# Autodesk Inventor assembly: XEndRight
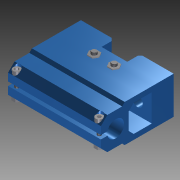
[picture p0: Inventor's stored thumbnail of the model, 180x180]
Saved by Autodesk Inventor 2015 (Build 190159000, 159)
## iProperties
Created: 2014-08-16
Part Number: XEndRight
Document SubType Name: Assembly
Designer: Jack
Author: Jack
## Documents named in this file (11)
- C:\Users\Jack\ownCloud\Projects\CoreXY\InventorModel\XAxis\DualE3DXEnd\XEndRight.iam
- C:\Users\Jack\ownCloud\Projects\CoreXY\InventorModel\XAxis\DualE3DXEnd\XEnd.ipt
- C:\Users\Jack\ownCloud\Projects\CoreXY\InventorModel\Hardware\Nuts\Nut3.ipt
- C:\Users\Jack\ownCloud\Projects\CoreXY\InventorModel\Hardware\Bolts\SHCS\SHCS3\SHCS3x18.ipt
- C:\Users\Jack\ownCloud\Projects\CoreXY\InventorModel\Hardware\Bolts\SHCS\SHCS4\SHCS4x30.ipt
- C:\Users\Jack\ownCloud\Projects\CoreXY\InventorModel\Hardware\Nuts\Nut4.ipt
- C:\Users\Jack\ownCloud\Projects\CoreXY\InventorModel\Hardware\Bearing\BearingRadialBall\BearingRadialBallF624zz.ipt
- C:\Users\Jack\ownCloud\Projects\CoreXY\InventorModel\Hardware\Wahsers\M4Washer.ipt
- C:\Users\Jack\ownCloud\Projects\CoreXY\InventorModel\Hardware\Bolts\SHCS\SHCS3\SHCS3x8.ipt
- C:\Users\Jack\ownCloud\Projects\CoreXY\InventorModel\XAxis\DualE3DXEnd\XAxisBearingSpacer.ipt
- C:\Users\Jack\ownCloud\Projects\CoreXY\InventorModel\Hardware\Bearing\BearingLinear\BearingLinearLMK8.ipt
## Components (25 placed, 10 different names)
1. XEnd:1 — Mate:5, Mate:6, Mate:7, Mate:8, Mate:9, Angle:1, Angle:2, Mate:10, Mate:11, Mate:13, Mate:15, Mate:16, Mate:17, Mate:18, Mate:19, Angle:3, Angle:4, Mate:22, Mate:23, Mate:40, Mate:41, Angle:5, Angle:6, Mate:44, Mate:45, Mate:46, Mate:47, Mate:62, Mate:63, Flush:3, Flush:4
2. XAxisBearingSpacer:1 — Mate:52, Mate:53
3. XAxisBearingSpacer:2 — Mate:54, Mate:55
4. BearingRadialBallF624zz:3
5. BearingRadialBallF624zz:4 — Mate:60, Mate:61
6. BearingLinearLMK8:1 — Mate:62, Flush:3
7. BearingLinearLMK8:2 — Mate:63, Flush:4
8. BearingRadialBallF624zz:1
9. BearingRadialBallF624zz:2
10. M4Washer:4 — Mate:38, Mate:46
11. M4Washer:3 — Mate:53, Mate:61
12. M4Washer:2 — Mate:30, Mate:55
13. M4Washer:1 — Mate:47
14. Nut4:2 — Mate:21, Angle:4, Mate:23
15. Nut4:1 — Mate:20, Angle:3, Mate:22
16. SHCS4x30:2 — Mate:17, Mate:18, Mate:20, Mate:38, Mate:52, Mate:60
17. SHCS4x30:1 — Mate:16, Mate:19, Mate:21, Mate:30, Mate:54
18. Nut3:3 — Mate:43, Angle:6, Mate:45, Flush:1
19. Nut3:4 — Mate:42, Angle:5, Mate:44, Flush:2
20. SHCS3x8:1 — Mate:40, Mate:42, Flush:2
21. SHCS3x8:2 — Mate:41, Mate:43, Flush:1
22. SHCS3x18:2 — Mate:14, Mate:15
23. SHCS3x18:1 — Mate:12, Mate:13
24. Nut3:2 — Mate:8, Angle:1, Mate:11, Mate:12
25. Nut3:1 — Mate:9, Angle:2, Mate:10, Mate:14
## Relationships (55: Mate 45, Angle 6, Flush 4)
- Mate:5: XEnd:1
- Mate:6: XEnd:1
- Mate:7: XEnd:1
- Mate:8: XEnd:1 ↔ Nut3:2
- Mate:9: XEnd:1 ↔ Nut3:1
- Angle:1 (0 deg): XEnd:1 ↔ Nut3:2
- Angle:2 (0 deg): XEnd:1 ↔ Nut3:1
- Mate:10: XEnd:1 ↔ Nut3:1
- Mate:11: XEnd:1 ↔ Nut3:2
- Mate:12: SHCS3x18:1 ↔ Nut3:2
- Mate:13: XEnd:1 ↔ SHCS3x18:1
- Mate:14: SHCS3x18:2 ↔ Nut3:1
- Mate:15: XEnd:1 ↔ SHCS3x18:2
- Mate:16: XEnd:1 ↔ SHCS4x30:1
- Mate:17: XEnd:1 ↔ SHCS4x30:2
- Mate:18: XEnd:1 ↔ SHCS4x30:2
- Mate:19: XEnd:1 ↔ SHCS4x30:1
- Mate:20: Nut4:1 ↔ SHCS4x30:2
- Mate:21: Nut4:2 ↔ SHCS4x30:1
- Angle:3 (0 deg): XEnd:1 ↔ Nut4:1
- Angle:4 (0 deg): XEnd:1 ↔ Nut4:2
- Mate:22: XEnd:1 ↔ Nut4:1
- Mate:23: XEnd:1 ↔ Nut4:2
- [Mate]: BearingRadialBallF624zz:1 ↔ BearingRadialBallF624zz:2
- [Mate]: BearingRadialBallF624zz:1 ↔ BearingRadialBallF624zz:2
- [Mate]: BearingRadialBallF624zz:1 ↔ M4Washer:1
- [Mate]: BearingRadialBallF624zz:1 ↔ M4Washer:1
- [Mate]: BearingRadialBallF624zz:2 ↔ M4Washer:2
- [Mate]: BearingRadialBallF624zz:2 ↔ M4Washer:2
- Mate:30: M4Washer:2 ↔ SHCS4x30:1
- Mate:38: M4Washer:4 ↔ SHCS4x30:2
- Mate:40: XEnd:1 ↔ SHCS3x8:1
- Mate:41: XEnd:1 ↔ SHCS3x8:2
- Mate:42: Nut3:4 ↔ SHCS3x8:1
- Mate:43: Nut3:3 ↔ SHCS3x8:2
- Angle:5 (0 deg): XEnd:1 ↔ Nut3:4
- Angle:6 (0 deg): XEnd:1 ↔ Nut3:3
- Mate:44: XEnd:1 ↔ Nut3:4
- Mate:45: XEnd:1 ↔ Nut3:3
- Flush:1 (-0.5 mm): Nut3:3 ↔ SHCS3x8:2
- Flush:2 (-0.5 mm): Nut3:4 ↔ SHCS3x8:1
- Mate:46: XEnd:1 ↔ M4Washer:4
- Mate:47: XEnd:1 ↔ M4Washer:1
- Mate:52: XAxisBearingSpacer:1 ↔ SHCS4x30:2
- Mate:53: XAxisBearingSpacer:1 ↔ M4Washer:3
- Mate:54: XAxisBearingSpacer:2 ↔ SHCS4x30:1
- Mate:55: XAxisBearingSpacer:2 ↔ M4Washer:2
- [Mate]: BearingRadialBallF624zz:3 ↔ BearingRadialBallF624zz:4
- [Mate]: BearingRadialBallF624zz:3 ↔ BearingRadialBallF624zz:4
- Mate:60: BearingRadialBallF624zz:4 ↔ SHCS4x30:2
- Mate:61: BearingRadialBallF624zz:4 ↔ M4Washer:3
- Mate:62: XEnd:1 ↔ BearingLinearLMK8:1
- Mate:63: XEnd:1 ↔ BearingLinearLMK8:2
- Flush:3: XEnd:1 ↔ BearingLinearLMK8:1
- Flush:4: XEnd:1 ↔ BearingLinearLMK8:2
## Named parameters: d85_d44 = 0 mm, d86_d45 = 0 mm
